# Autodesk Inventor assembly: s-assy-unit-gear
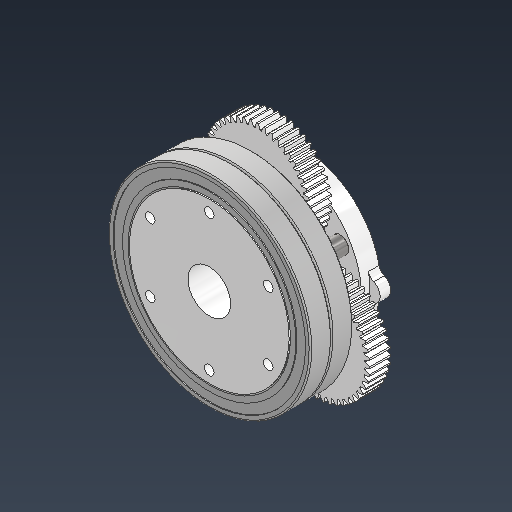
[picture p0: Inventor's stored thumbnail of the model, 512x512]
Saved by Autodesk Inventor 2021 (Build 250183000, 183)
## iProperties
Created: 2021-07-12
Part Number: s-assy-unit-gear
Document SubType Name: Assembly
Designer: yuta0
Author: yuta0
## Documents named in this file (10)
- C:\Users\yuta0\Desktop\catchrobo_robot\s-assy-unit-gear.iam
- C:\Users\yuta0\Desktop\catchrobo_robot\base24.ipt
- C:\Users\yuta0\Desktop\catchrobo_robot\B6808ZZ.ipt
- C:\Users\yuta0\Desktop\catchrobo_robot\ARF-413E.ipt
- C:\Users\yuta0\Desktop\catchrobo_robot\s-assy-unit-planet_gear.iam
- C:\Users\yuta0\Desktop\catchrobo_robot\CBSTSR4-14.ipt
- C:\Users\yuta0\Desktop\catchrobo_robot\carbon_plate11.ipt
- C:\Users\yuta0\Desktop\catchrobo_robot\B6815ZZ.ipt
- C:\Users\yuta0\Desktop\catchrobo_robot\base25.ipt
- C:\Users\yuta0\Desktop\catchrobo_robot\B6901ZZ.ipt
## Components (22 placed, 9 different names)
1. unit-base1:1 — メイト:1, メイト:2, メイト:3, メイト:4, メイト:6, メイト:7, メイト:8
2. B6808ZZ:1 — メイト:1, メイト:2
3. unit-plate1:1 — メイト:9, メイト:10, メイト:11, メイト:12, メイト:13, メイト:17, メイト:18
4. B6815ZZ:1 — メイト:12, メイト:13, メイト:14, メイト:15
5. B6815ZZ:2 — メイト:14, メイト:15, メイト:16
6. unit-base2:1 — メイト:16, メイト:17, メイト:18, メイト:22, メイト:23
7. B6901ZZ:1 — メイト:22, メイト:23
8. unir-spacer1:1 — メイト:3, メイト:4, メイト:5, メイト:9, メイト:10
9. CBSTSR4-14:1 — メイト:7, メイト:8
10. unir-spacer1:2
11. CBSTSR4-14:2
12. unir-spacer1:3
13. CBSTSR4-14:3
14. unir-spacer1:4
15. CBSTSR4-14:4
16. unir-spacer1:5
17. CBSTSR4-14:5
18. unir-spacer1:6
19. CBSTSR4-14:6
20. s-assy-unit-planet_gear:1 [sub-assembly] — メイト:5, メイト:6
21. s-assy-unit-planet_gear:2 [sub-assembly]
22. s-assy-unit-planet_gear:3 [sub-assembly]
## Component patterns: (6 elements, first: unir-spacer1:1 + CBSTSR4-14:1), (3 elements, first: s-assy-unit-planet_gear:1)
## Relationships (20: Mate 20)
- メイト:1 [Mate]: unit-base1:1 ↔ B6808ZZ:1
- メイト:2 [Mate]: unit-base1:1 ↔ B6808ZZ:1
- メイト:3 [Mate]: unit-base1:1 ↔ unir-spacer1:1
- メイト:4 [Mate]: unit-base1:1 ↔ unir-spacer1:1
- メイト:5 [Mate]: unir-spacer1:1 ↔ s-assy-unit-planet_gear:1
- メイト:6 [Mate]: unit-base1:1 ↔ s-assy-unit-planet_gear:1
- メイト:7 [Mate]: unit-base1:1 ↔ CBSTSR4-14:1
- メイト:8 [Mate]: unit-base1:1 ↔ CBSTSR4-14:1
- メイト:9 [Mate]: unit-plate1:1 ↔ unir-spacer1:1
- メイト:10 [Mate]: unit-plate1:1 ↔ unir-spacer1:1
- メイト:11 [Mate]: unit-plate1:1
- メイト:12 [Mate]: unit-plate1:1 ↔ B6815ZZ:1
- メイト:13 [Mate]: unit-plate1:1 ↔ B6815ZZ:1
- メイト:14 [Mate]: B6815ZZ:1 ↔ B6815ZZ:2
- メイト:15 [Mate]: B6815ZZ:1 ↔ B6815ZZ:2
- メイト:16 [Mate]: B6815ZZ:2 ↔ unit-base2:1
- メイト:17 [Mate]: unit-plate1:1 ↔ unit-base2:1
- メイト:18 [Mate]: unit-plate1:1 ↔ unit-base2:1
- メイト:22 [Mate]: unit-base2:1 ↔ B6901ZZ:1
- メイト:23 [Mate]: unit-base2:1 ↔ B6901ZZ:1
